# Autodesk Inventor assembly: baza
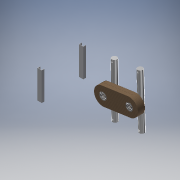
[picture p0: Inventor's stored thumbnail of the model, 180x180]
Saved by Autodesk Inventor 2017 (Build 210142000, 142)
## iProperties
Part Number: baza
Material: Ogólny
Document SubType Name: Assembly
Designer: Dorota
Author: Dorota
## Documents named in this file (5)
- C:\Users\Dorota\Downloads\rudder\rudder\baza.iam
- C:\Users\Dorota\Downloads\rudder\rudder\palak.iam
- C:\Users\Dorota\Downloads\rudder\rudder\podstawa.ipt
- C:\Users\Dorota\Downloads\rudder\rudder\baza\Design Accelerator\Łożysko1.iam
- C:\Users\Dorota\Downloads\rudder\rudder\ceownik.ipt
## Components (10 placed, 4 different names)
1. palak:1 [sub-assembly] — Równoległy:1, Zestawiający:14, Zestawiający:15
2. podstawa:1 — Zestawiający:1, Zestawiający:2, Zestawiający:3, Zestawiający:5, Zestawiający:6, Zestawiający:7, Zestawiający:8
3. palak:2 [sub-assembly] — Równoległy:1, Zestawiający:13
4. podstawa:2 — Zestawiający:1, Zestawiający:2, Zestawiający:3, Zestawiający:4, Zestawiający:11, Zestawiający:12
5. Łożysko:1 [sub-assembly] — Zestawiający:5, Zestawiający:6, Zestawiający:10, Zestawiający:13
6. Łożysko:2 [sub-assembly] — Zestawiający:9, Zestawiający:11
7. Łożysko:3 [sub-assembly] — Zestawiający:10, Zestawiający:12
8. Łożysko:4 [sub-assembly] — Zestawiający:7, Zestawiający:8, Zestawiający:9, Zestawiający:14, Zestawiający:15
9. ceownik:1 — Równoległy:2
10. ceownik:2 — Równoległy:2
## Relationships (17: Mate 15, Flush 2)
- Zestawiający:1 [Mate]: podstawa:1 ↔ podstawa:2
- Zestawiający:2 [Mate]: podstawa:1 ↔ podstawa:2
- Zestawiający:3 [Mate]: podstawa:1 ↔ podstawa:2
- Zestawiający:4 [Mate]: podstawa:2
- Równoległy:1 [Flush]: palak:1 ↔ palak:2
- Zestawiający:5 [Mate]: podstawa:1 ↔ Łożysko:1
- Zestawiający:6 [Mate]: podstawa:1 ↔ Łożysko:1
- Zestawiający:7 [Mate]: podstawa:1 ↔ Łożysko:4
- Zestawiający:8 [Mate]: podstawa:1 ↔ Łożysko:4
- Zestawiający:9 [Mate]: Łożysko:2 ↔ Łożysko:4
- Zestawiający:10 [Mate]: Łożysko:1 ↔ Łożysko:3
- Zestawiający:11 [Mate]: podstawa:2 ↔ Łożysko:2
- Zestawiający:12 [Mate]: podstawa:2 ↔ Łożysko:3
- Zestawiający:13 [Mate]: palak:2 ↔ Łożysko:1
- Zestawiający:14 [Mate]: palak:1 ↔ Łożysko:4
- Zestawiający:15 [Mate]: palak:1 ↔ Łożysko:4
- Równoległy:2 [Flush]: ceownik:1 ↔ ceownik:2
